# Autodesk Inventor assembly: VersaRoller Generator
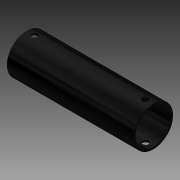
[picture p0: Inventor's stored thumbnail of the model, 180x180]
Saved by Autodesk Inventor 2022 (Build 260153000, 153)
## iProperties
Created: 2021-08-02
Part Number: VersaRoller Generator
Document SubType Name: Assembly
## Documents named in this file (3)
- C:\Users\Cal\Desktop\Robotics\Design\Collaborative\Collaborative Parts Library\Wheels and Rollers\Roller Parts\VersaRoller Generator.iam
- C:\Users\Cal\Desktop\Robotics\Design\Collaborative\Collaborative Parts Library\Wheels and Rollers\Roller Parts\Versa Tube Generator\4 in Versa Tube.ipt
- C:\Users\Cal\Desktop\Robotics\Design\Collaborative\Collaborative Parts Library\Wheels and Rollers\Roller Parts\VersaTube Generator.ipt
## Components (1 placed, 1 different names)
1. 4 in Versa Tube:1
## Named parameters: VersaTubeLength = 101.6 mm, VersaTubeInput = 25.4 mm
